# Autodesk Inventor assembly: ramaGusenitsi
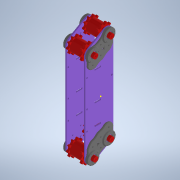
[picture p0: Inventor's stored thumbnail of the model, 180x180]
Saved by Autodesk Inventor 2020 (Build 240168000, 168)
## iProperties
Created: 2022-10-22
Part Number: ramaGusenitsi
Document SubType Name: Assembly
Designer: Inventor-2
Author: Inventor-2
## Documents named in this file (6)
- C:\Projects\AndruXD\Sborki\ramaGusenitsi.iam
- C:\Projects\AndruXD\stenka.ipt
- C:\Projects\AndruXD\kolesoIn.ipt
- C:\Projects\AndruXD\kolesoOut.ipt
- C:\Projects\AndruXD\korpusPodshipnika.ipt
- C:\Projects\AndruXD\korpusPodshipnika1.ipt
## Components (14 placed, 4 different names)
1. stenka:1 — Заподлицо:1, Заподлицо:2, Совмещение:13, Совмещение:14, Совмещение:15, Совмещение:16, Совмещение:18, Совмещение:27
2. stenka:2 — Совмещение:9, Совмещение:10, Совмещение:11, Совмещение:12, Заподлицо:1, Заподлицо:2, Совмещение:21, Совмещение:24
3. kolesoIn:1 — Совмещение:4, Совмещение:16, Совмещение:19
4. kolesoIn:2 — Совмещение:3, Совмещение:15, Совмещение:20
5. kolesoIn:3 — Совмещение:2, Совмещение:14, Совмещение:28
6. kolesoIn:4 — Совмещение:1, Совмещение:13, Совмещение:29
7. kolesoOut:1 — Совмещение:4, Совмещение:12, Совмещение:26
8. kolesoOut:2 — Совмещение:3, Совмещение:11, Совмещение:25
9. kolesoOut:3 — Совмещение:2, Совмещение:10, Совмещение:23
10. kolesoOut:4 — Совмещение:1, Совмещение:9, Совмещение:22
11. korpusPodshipnika:1 — Совмещение:27, Совмещение:28, Совмещение:29
12. korpusPodshipnika:2 — Совмещение:18, Совмещение:19, Совмещение:20
13. korpusPodshipnika:3 — Совмещение:21, Совмещение:22, Совмещение:23
14. korpusPodshipnika:4 — Совмещение:24, Совмещение:25, Совмещение:26
## Relationships (26: Mate 24, Flush 2)
- Совмещение:1 [Mate]: kolesoIn:4 ↔ kolesoOut:4
- Совмещение:2 [Mate]: kolesoIn:3 ↔ kolesoOut:3
- Совмещение:3 [Mate]: kolesoIn:2 ↔ kolesoOut:2
- Совмещение:4 [Mate]: kolesoIn:1 ↔ kolesoOut:1
- Совмещение:9 [Mate]: stenka:2 ↔ kolesoOut:4
- Совмещение:10 [Mate]: stenka:2 ↔ kolesoOut:3
- Совмещение:11 [Mate]: stenka:2 ↔ kolesoOut:2
- Совмещение:12 [Mate]: stenka:2 ↔ kolesoOut:1
- Заподлицо:1 [Flush]: stenka:1 ↔ stenka:2
- Заподлицо:2 [Flush]: stenka:1 ↔ stenka:2
- Совмещение:13 [Mate]: stenka:1 ↔ kolesoIn:4
- Совмещение:14 [Mate]: stenka:1 ↔ kolesoIn:3
- Совмещение:15 [Mate]: stenka:1 ↔ kolesoIn:2
- Совмещение:16 [Mate]: stenka:1 ↔ kolesoIn:1
- Совмещение:18 [Mate]: stenka:1 ↔ korpusPodshipnika:2
- Совмещение:19 [Mate]: kolesoIn:1 ↔ korpusPodshipnika:2
- Совмещение:20 [Mate]: kolesoIn:2 ↔ korpusPodshipnika:2
- Совмещение:21 [Mate]: stenka:2 ↔ korpusPodshipnika:3
- Совмещение:22 [Mate]: kolesoOut:4 ↔ korpusPodshipnika:3
- Совмещение:23 [Mate]: kolesoOut:3 ↔ korpusPodshipnika:3
- Совмещение:24 [Mate]: stenka:2 ↔ korpusPodshipnika:4
- Совмещение:25 [Mate]: kolesoOut:2 ↔ korpusPodshipnika:4
- Совмещение:26 [Mate]: kolesoOut:1 ↔ korpusPodshipnika:4
- Совмещение:27 [Mate]: stenka:1 ↔ korpusPodshipnika:1
- Совмещение:28 [Mate]: kolesoIn:3 ↔ korpusPodshipnika:1
- Совмещение:29 [Mate]: kolesoIn:4 ↔ korpusPodshipnika:1
